# Autodesk Inventor assembly: Shooter_Flywheel
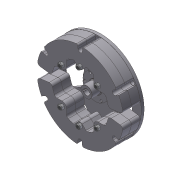
[picture p0: Inventor's stored thumbnail of the model, 180x180]
Saved by Autodesk Inventor 2012 (Build 160160000, 160)
## iProperties
Created: 2012-01-29
Part Number: Shooter_Flywheel
Document SubType Name: Assembly
Designer: JesseK
Mass: 2027.9 g
Surface Area: 1790.83 cm^2
Volume: 737.239 cm^3
Density: 2.75066 g/cm^3
Author: JesseK
## Documents named in this file (6)
- Z:\UserData\Documents\Inventor\team1885frc\Robot2012\Shooter\Shooter_Flywheel.iam
- Z:\UserData\Documents\Inventor\team1885frc\Robot2012\Shooter\FlyWheel_Base_Jan21.ipt
- Z:\UserData\Documents\Inventor\team1885frc\Robot2012\Shooter\IFI_Wheel_Weight_8in.ipt
- Z:\UserData\Documents\Inventor\team1885frc\Hardware\Bolts\Bolt_Num10_32_2.0len_SocketHead.ipt
- Z:\UserData\Documents\Inventor\team1885frc\Hardware\Nuts\LockNut_Num10_32.ipt
- Z:\UserData\Documents\Inventor\team1885frc\AndyMark\500EX-Key-Hub.ipt
## Components (18 placed, 5 different names)
1. FlyWheel_Base_Jan21:1 — Mate:1, Mate:2, Mate:5, Mate:6, Mate:9, Mate:10, Mate:19, Mate:20, Mate:21, Mate:22, Mate:23, Mate:24, Mate:37, Mate:38, Mate:39
2. IFI_Wheel_Weight_8in:1 — Mate:2, Mate:3, Mate:5, Mate:6, Mate:7, Mate:8
3. IFI_Wheel_Weight_8in:2 — Mate:1, Mate:4, Mate:9, Mate:10, Mate:11, Mate:12
4. IFI_Wheel_Weight_8in:3 — Mate:3, Mate:7, Mate:8, Mate:13, Mate:14, Mate:15, Mate:25, Mate:26, Mate:27
5. IFI_Wheel_Weight_8in:4 — Mate:4, Mate:11, Mate:12, Mate:16, Mate:17, Mate:18, Mate:28, Mate:29, Mate:30
6. Bolt_Num10_32_2.0len_SocketHead:1 — Mate:16, Mate:19, Mate:33
7. Bolt_Num10_32_2.0len_SocketHead:2 — Mate:17, Mate:20, Mate:32
8. Bolt_Num10_32_2.0len_SocketHead:3 — Mate:18, Mate:24, Mate:31
9. Bolt_Num10_32_2.0len_SocketHead:4 — Mate:15, Mate:21, Mate:34
10. Bolt_Num10_32_2.0len_SocketHead:5 — Mate:14, Mate:22, Mate:35
11. Bolt_Num10_32_2.0len_SocketHead:6 — Mate:13, Mate:23, Mate:36
12. LockNut_Num10_32:1 — Mate:25, Mate:36
13. LockNut_Num10_32:2 — Mate:26, Mate:35
14. LockNut_Num10_32:3 — Mate:27, Mate:34
15. LockNut_Num10_32:4 — Mate:28, Mate:31
16. LockNut_Num10_32:5 — Mate:30, Mate:32
17. LockNut_Num10_32:6 — Mate:29, Mate:33
18. 500EX-Key-Hub:1 — Mate:37, Mate:38, Mate:39
## Relationships (39: Mate 39)
- Mate:1: FlyWheel_Base_Jan21:1 ↔ IFI_Wheel_Weight_8in:2
- Mate:2: FlyWheel_Base_Jan21:1 ↔ IFI_Wheel_Weight_8in:1
- Mate:3: IFI_Wheel_Weight_8in:1 ↔ IFI_Wheel_Weight_8in:3
- Mate:4: IFI_Wheel_Weight_8in:2 ↔ IFI_Wheel_Weight_8in:4
- Mate:5: FlyWheel_Base_Jan21:1 ↔ IFI_Wheel_Weight_8in:1
- Mate:6: FlyWheel_Base_Jan21:1 ↔ IFI_Wheel_Weight_8in:1
- Mate:7: IFI_Wheel_Weight_8in:1 ↔ IFI_Wheel_Weight_8in:3
- Mate:8: IFI_Wheel_Weight_8in:1 ↔ IFI_Wheel_Weight_8in:3
- Mate:9: FlyWheel_Base_Jan21:1 ↔ IFI_Wheel_Weight_8in:2
- Mate:10: FlyWheel_Base_Jan21:1 ↔ IFI_Wheel_Weight_8in:2
- Mate:11: IFI_Wheel_Weight_8in:2 ↔ IFI_Wheel_Weight_8in:4
- Mate:12: IFI_Wheel_Weight_8in:2 ↔ IFI_Wheel_Weight_8in:4
- Mate:13: IFI_Wheel_Weight_8in:3 ↔ Bolt_Num10_32_2.0len_SocketHead:6
- Mate:14: IFI_Wheel_Weight_8in:3 ↔ Bolt_Num10_32_2.0len_SocketHead:5
- Mate:15: IFI_Wheel_Weight_8in:3 ↔ Bolt_Num10_32_2.0len_SocketHead:4
- Mate:16: IFI_Wheel_Weight_8in:4 ↔ Bolt_Num10_32_2.0len_SocketHead:1
- Mate:17: IFI_Wheel_Weight_8in:4 ↔ Bolt_Num10_32_2.0len_SocketHead:2
- Mate:18: IFI_Wheel_Weight_8in:4 ↔ Bolt_Num10_32_2.0len_SocketHead:3
- Mate:19: FlyWheel_Base_Jan21:1 ↔ Bolt_Num10_32_2.0len_SocketHead:1
- Mate:20: FlyWheel_Base_Jan21:1 ↔ Bolt_Num10_32_2.0len_SocketHead:2
- Mate:21: FlyWheel_Base_Jan21:1 ↔ Bolt_Num10_32_2.0len_SocketHead:4
- Mate:22: FlyWheel_Base_Jan21:1 ↔ Bolt_Num10_32_2.0len_SocketHead:5
- Mate:23: FlyWheel_Base_Jan21:1 ↔ Bolt_Num10_32_2.0len_SocketHead:6
- Mate:24: FlyWheel_Base_Jan21:1 ↔ Bolt_Num10_32_2.0len_SocketHead:3
- Mate:25: IFI_Wheel_Weight_8in:3 ↔ LockNut_Num10_32:1
- Mate:26: IFI_Wheel_Weight_8in:3 ↔ LockNut_Num10_32:2
- Mate:27: IFI_Wheel_Weight_8in:3 ↔ LockNut_Num10_32:3
- Mate:28: IFI_Wheel_Weight_8in:4 ↔ LockNut_Num10_32:4
- Mate:29: IFI_Wheel_Weight_8in:4 ↔ LockNut_Num10_32:6
- Mate:30: IFI_Wheel_Weight_8in:4 ↔ LockNut_Num10_32:5
- Mate:31: Bolt_Num10_32_2.0len_SocketHead:3 ↔ LockNut_Num10_32:4
- Mate:32: Bolt_Num10_32_2.0len_SocketHead:2 ↔ LockNut_Num10_32:5
- Mate:33: Bolt_Num10_32_2.0len_SocketHead:1 ↔ LockNut_Num10_32:6
- Mate:34: Bolt_Num10_32_2.0len_SocketHead:4 ↔ LockNut_Num10_32:3
- Mate:35: Bolt_Num10_32_2.0len_SocketHead:5 ↔ LockNut_Num10_32:2
- Mate:36: Bolt_Num10_32_2.0len_SocketHead:6 ↔ LockNut_Num10_32:1
- Mate:37: FlyWheel_Base_Jan21:1 ↔ 500EX-Key-Hub:1
- Mate:38: FlyWheel_Base_Jan21:1 ↔ 500EX-Key-Hub:1
- Mate:39: FlyWheel_Base_Jan21:1 ↔ 500EX-Key-Hub:1
